# Autodesk Inventor assembly: Outer_support_stand_WearingImage
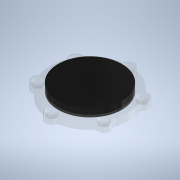
[picture p0: Inventor's stored thumbnail of the model, 180x180]
Saved by Autodesk Inventor 2020.4 (Build 244396000, 396)
## iProperties
Created: 2022-03-16
Part Number: Outer_support_stand_WearingImage
Document SubType Name: Assembly
Designer: Masato Kubotera
Author: Masato Kubotera
## Documents named in this file (3)
- C:\Users\Masato\Documents\Inventor\CIT Brains_Inventor\SUSTAINA-OP\SandBlastingJig\Outer_support_stand_WearingImage.iam
- C:\Users\Masato\Documents\Inventor\CIT Brains_Inventor\SUSTAINA-OP\UpperBody\Trunk\CrossRollerBearing\Outer_support_stand.ipt
- C:\Users\Masato\Documents\Inventor\CIT Brains_Inventor\SUSTAINA-OP\SandBlastingJig\Outer_support_stand_SandBlastingJig.ipt
## Components (2 placed, 2 different names)
1. Outer_support_stand:1 — 挿入:1
2. Outer_support_stand_SandBlastingJig:1 — 挿入:1
## Relationships (1: Insert 1)
- 挿入:1 [Insert]: Outer_support_stand:1 ↔ Outer_support_stand_SandBlastingJig:1
